# Autodesk Inventor assembly: W13-4
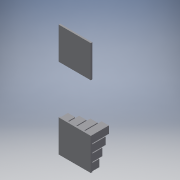
[picture p0: Inventor's stored thumbnail of the model, 180x180]
Saved by Autodesk Inventor 2017 (Build 210142000, 142)
## iProperties
Created: 2020-12-29
Part Number: W13-4
Material: 一般
Document SubType Name: Assembly
Designer: Brian
Sending System: Autodesk Inventor 2020
Preprocessor: ST-DEVELOPER v18
Title: F:\DesktopSpace\MASTERS\ma2010_asm.stp
Author: Crowm
Revision Number: ANY
## Documents named in this file (3)
- E:\coppeliaSim\3D\機械手臂 3D\W13-4.iam
- E:\coppeliaSim\3D\機械手臂 3D\底座.ipt
- E:\coppeliaSim\3D\機械手臂 3D\方塊.ipt
## Components (3 placed, 2 different names)
1. 底座:1 — Flush:3, Flush:4, Mate:33, Mate:34, Flush:5, Flush:6
2. 底座:2 — Flush:3, Flush:4, Mate:33
3. 方塊:1 — Mate:34, Flush:5, Flush:6
## Relationships (6: Flush 4, Mate 2)
- Flush:3: 底座:1 ↔ 底座:2
- Flush:4: 底座:1 ↔ 底座:2
- Mate:33 (600 mm): 底座:1 ↔ 底座:2
- Mate:34: 底座:1 ↔ 方塊:1
- Flush:5 (-5 mm): 底座:1 ↔ 方塊:1
- Flush:6 (-5 mm): 底座:1 ↔ 方塊:1
